# Autodesk Inventor assembly: pcb_btm
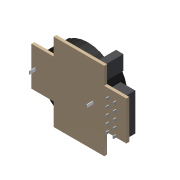
[picture p0: Inventor's stored thumbnail of the model, 180x180]
Saved by Autodesk Inventor 2015 SP1 (Build 190203100, 203)
## iProperties
Created: 2015-12-08
Part Number: pcb_btm
Document SubType Name: Assembly
Designer: User
Mass: 0.99462 g
Surface Area: 21.1298 cm^2
Volume: 1.02765 cm^3
Density: 0.967858 g/cm^3
Author: User
## Documents named in this file (5)
- C:\Users\User\Downloads\kurs_mark\Inventor\pcb_btm.iam
- C:\Users\User\Downloads\kurs_mark\Inventor\pcb_btm.ipt
- C:\Users\User\Downloads\kurs_mark\Inventor\bs-7.ipt
- C:\Users\User\Downloads\kurs_mark\Inventor\jumper.ipt
- C:\Users\User\Downloads\kurs_mark\Inventor\MOLEX.ipt
## Components (4 placed, 4 different names)
1. pcb_btm:1 — Заподлицо:1, Совмещение:1, Совмещение:2
2. bs-7:1 — Заподлицо:1
3. jumper:1 — Совмещение:1
4. MOLEX:1 — Совмещение:2
## Relationships (3: Mate 2, Flush 1)
- Заподлицо:1 [Flush] (0.4 mm): pcb_btm:1 ↔ bs-7:1
- Совмещение:1 [Mate]: pcb_btm:1 ↔ jumper:1
- Совмещение:2 [Mate]: pcb_btm:1 ↔ MOLEX:1
